# Autodesk Inventor assembly: 2AM-17-A-4200 - inside slider
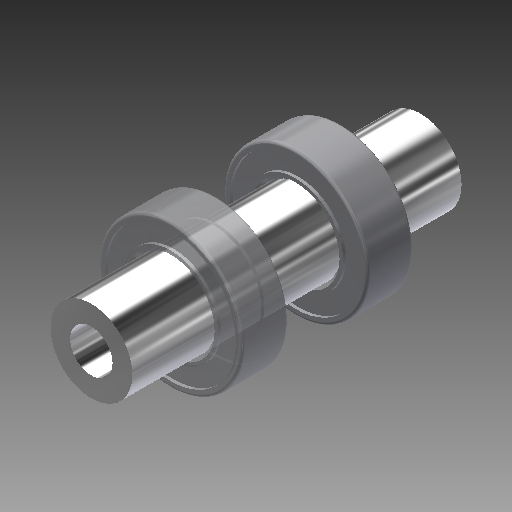
[picture p0: Inventor's stored thumbnail of the model, 512x512]
Saved by Autodesk Inventor 2017 (Build 210142000, 142)
## iProperties
Created: 2017-12-27
Part Number: 2AM-17-A-4200 - inside slider
Document SubType Name: Assembly
Designer: Micah
Mass: 39.4981 g
Surface Area: 59.6025 cm^2
Volume: 8.09562 cm^3
Density: 4.87894 g/cm^3
Author: Micah
## Documents named in this file (3)
- C:\Users\Micah\Desktop\inventor\CADathon-2017\2AM-17-A-0200 - Smokestack Elevator\2AM-17-A-4200 - inside slider.iam
- C:\Users\Micah\Desktop\inventor\CADathon-2017\2AM-17-A-0200 - Smokestack Elevator\COTS\0_500_ID_x_0_875_OD_x_0_281_WD_Radial_Bearing_217-3337.ipt
- C:\Users\Micah\Desktop\inventor\CADathon-2017\2AM-17-A-0200 - Smokestack Elevator\2AM-17-P-4201 - tube shaft.ipt
## Components (3 placed, 2 different names)
1. 0_500_ID_x_0_875_OD_x_0_281_WD_Radial_Bearing_217-3337:1 — Rotational:1
2. 0_500_ID_x_0_875_OD_x_0_281_WD_Radial_Bearing_217-3337:2 — Rotational:2
3. 2AM-17-P-4201 - tube shaft:1 — Rotational:1, Rotational:2
## Relationships (2: RevoluteJoint 2)
- Rotational:1 [RevoluteJoint] (-12.192 mm): 0_500_ID_x_0_875_OD_x_0_281_WD_Radial_Bearing_217-3337:1 ↔ 2AM-17-P-4201 - tube shaft:1
- Rotational:2 [RevoluteJoint] (-12.192 mm): 0_500_ID_x_0_875_OD_x_0_281_WD_Radial_Bearing_217-3337:2 ↔ 2AM-17-P-4201 - tube shaft:1
